# Autodesk Inventor assembly: 75mm Mecanum Wheel Set
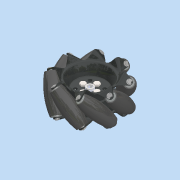
[picture p0: Inventor's stored thumbnail of the model, 180x180]
Saved by Autodesk Inventor 2022 (Build 260153000, 153)
## iProperties
Created: 2019-09-10
Part Number: 75mm Mecanum Wheel Set
Description: STEP AP214
Document SubType Name: Assembly
Designer: izack
Sending System: SolidWorks 2018
Preprocessor: SwSTEP 2.0
Title: REV-41-1656.STEP
Revision Number: ANY
## Documents named in this file (8)
- E:\saji_john\Documents\GitHub\ComputerAidedDesign\2021-22\FTC\#13822 Robovikes\Proof of Concept\13in^3 drivetrain parts\75mm Mecanum Wheel Set.iam
- E:\saji_john\Documents\GitHub\ComputerAidedDesign\2021-22\FTC\#13822 Robovikes\Proof of Concept\13in^3 drivetrain parts\75mm Mecanum Wheel Set\REV-41-1656-1.ipt
- E:\saji_john\Documents\GitHub\ComputerAidedDesign\2021-22\FTC\#13822 Robovikes\Proof of Concept\13in^3 drivetrain parts\75mm Mecanum Wheel Set\REV-41-1656-2.ipt
- E:\saji_john\Documents\GitHub\ComputerAidedDesign\2021-22\FTC\#13822 Robovikes\Proof of Concept\13in^3 drivetrain parts\75mm Mecanum Wheel Set\REV-41-1655-3.iam
- E:\saji_john\Documents\GitHub\ComputerAidedDesign\2021-22\FTC\#13822 Robovikes\Proof of Concept\13in^3 drivetrain parts\75mm Mecanum Wheel Set\REV-41-1655-4 Assembly.iam
- E:\saji_john\Documents\GitHub\ComputerAidedDesign\2021-22\FTC\#13822 Robovikes\Proof of Concept\13in^3 drivetrain parts\75mm Mecanum Wheel Set\REV-41-1216.ipt
- E:\saji_john\Documents\GitHub\ComputerAidedDesign\2021-22\FTC\#13822 Robovikes\Proof of Concept\13in^3 drivetrain parts\75mm Mecanum Wheel Set\REV-41-1359 Simple.ipt
- E:\saji_john\Documents\GitHub\ComputerAidedDesign\2021-22\FTC\Parts\REV Parts\Hex Hub Adapter - 2 Pack.ipt
## Components (24 placed, 24 different names)
1. REV-41-1656-1_1 — Mate:1, Mate:2, Mate:4
2. REV-41-1656-2_2
3. REV-41-1655-3_3 [sub-assembly]
4. REV-41-1655-4 Assembly_4 [sub-assembly]
5. REV-41-1655-3_5 [sub-assembly]
6. REV-41-1655-3_6 [sub-assembly]
7. REV-41-1655-3_7 [sub-assembly]
8. REV-41-1655-3_8 [sub-assembly]
9. REV-41-1655-3_9 [sub-assembly]
10. REV-41-1655-3_10 [sub-assembly]
11. REV-41-1655-3_11 [sub-assembly]
12. REV-41-1655-4 Assembly_12 [sub-assembly]
13. REV-41-1655-4 Assembly_13 [sub-assembly]
14. REV-41-1655-4 Assembly_14 [sub-assembly]
15. REV-41-1655-4 Assembly_15 [sub-assembly]
16. REV-41-1655-4 Assembly_16 [sub-assembly]
17. REV-41-1655-4 Assembly_17 [sub-assembly]
18. REV-41-1655-4 Assembly_18 [sub-assembly]
19. REV-41-1216_19
20. REV-41-1359 Simple_20
21. REV-41-1359 Simple_21
22. REV-41-1359 Simple_22 — Mate:3, Mate:4
23. REV-41-1359 Simple_23
24. Hex Hub Adapter - 2 Pack:1 — Mate:1, Mate:2, Mate:3
## Relationships (4: Mate 4)
- Mate:1: REV-41-1656-1_1 ↔ Hex Hub Adapter - 2 Pack:1
- Mate:2: REV-41-1656-1_1 ↔ Hex Hub Adapter - 2 Pack:1
- Mate:3: REV-41-1359 Simple_22 ↔ Hex Hub Adapter - 2 Pack:1
- Mate:4: REV-41-1656-1_1 ↔ REV-41-1359 Simple_22
